# Autodesk Inventor assembly: gears
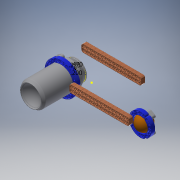
[picture p0: Inventor's stored thumbnail of the model, 180x180]
Saved by Autodesk Inventor 2019.3 (Build 233278000, 278)
## iProperties
Created: 2019-01-24
Part Number: gears
Document SubType Name: Assembly
Designer: Varga Daniel
Author: Varga Daniel
## Documents named in this file (9)
- C:\!_Dani\!_cloud\OneDrive\!_munka\Revolution\RevvyDemoKit\Structural parts\Part_test_Assembly.iam
- C:\!_Dani\!_cloud\OneDrive\!_munka\Revolution\RevvyDemoKit\Structural parts\Beams\Straight Beams\S2+x2\S16x2.iam
- C:\!_Dani\!_cloud\OneDrive\!_munka\Revolution\RevvyDemoKit\Structural parts\Beams\Straight Beams\S2+x2.iam
- C:\!_Dani\!_cloud\OneDrive\!_munka\Revolution\RevvyDemoKit\Structural parts\Beams\Curved beams\CB4H.ipt
- C:\!_Dani\!_cloud\OneDrive\!_munka\Revolution\RevvyDemoKit\Structural parts\Beams\Curved beams\CB6H.ipt
- C:\!_Dani\!_cloud\OneDrive\!_munka\Revolution\RevvyDemoKit\Structural parts\Beams\Curved beams\cocacola can.ipt
- C:\!_Dani\!_cloud\OneDrive\!_munka\Revolution\RevvyDemoKit\Structural parts\Beams\Straight Beams\S2+x1\S2x1.iam
- C:\!_Dani\!_cloud\OneDrive\!_munka\Revolution\RevvyDemoKit\Structural parts\Beams\Straight Beams\S2+x1.iam
- C:\!_Dani\!_cloud\OneDrive\!_munka\Revolution\RevvyDemoKit\Structural parts\Beams\Curved beams\Table tennis ball.ipt
## Components (14 placed, 6 different names)
1. S16x2:1 [sub-assembly] — Mate:1, Mate:2, Mate:3, Mate:4, Mate:14, Mate:15, Mate:16, Mate:17, Mate:25, Mate:26
2. S16x2:2 [sub-assembly]
3. CB4H:1 — Mate:14, Mate:15, Mate:19, Mate:26, Tangent:1
4. CB6H:1 — Mate:1, Mate:2, Mate:6, Mate:12, Mate:13
5. cocacola can:1 — Mate:5, Flush:1, Mate:6, Mate:11
6. CB6H:2 — Mate:3, Mate:4, Mate:5, Flush:1, Mate:9, Mate:10
7. S2x1:1 [sub-assembly] — Mate:7, Mate:8, Mate:9, Mate:10
8. S2x1:2 [sub-assembly] — Mate:12, Mate:13, Tangent:2
9. S2x1:3 [sub-assembly] — Mate:22, Mate:23, Mate:24
10. CB6H:3 — Mate:7, Mate:8, Mate:11, Tangent:2
11. Table tennis ball:1 — Mate:18, Mate:19, Mate:20, Mate:21
12. CB4H:2 — Mate:16, Mate:17, Mate:18, Mate:21, Flush:2, Mate:22, Mate:23, Mate:25
13. CB4H:3 — Mate:20, Flush:2, Mate:24, Mate:27, Mate:28
14. S2x1:4 [sub-assembly] — Mate:27, Mate:28, Tangent:1
## Relationships (32: Mate 28, Flush 2, Tangent 2)
- Mate:1: S16x2:1 ↔ CB6H:1
- Mate:2: S16x2:1 ↔ CB6H:1
- Mate:3: S16x2:1 ↔ CB6H:2
- Mate:4: S16x2:1 ↔ CB6H:2
- Mate:5: cocacola can:1 ↔ CB6H:2
- Flush:1 (-30 mm): cocacola can:1 ↔ CB6H:2
- Mate:6: CB6H:1 ↔ cocacola can:1
- Mate:7: S2x1:1 ↔ CB6H:3
- Mate:8: S2x1:1 ↔ CB6H:3
- Mate:9: CB6H:2 ↔ S2x1:1
- Mate:10: CB6H:2 ↔ S2x1:1
- Mate:11: cocacola can:1 ↔ CB6H:3
- Mate:12: CB6H:1 ↔ S2x1:2
- Mate:13: CB6H:1 ↔ S2x1:2
- Mate:14: S16x2:1 ↔ CB4H:1
- Mate:15: S16x2:1 ↔ CB4H:1
- Mate:16: S16x2:1 ↔ CB4H:2
- Mate:17: S16x2:1 ↔ CB4H:2
- Mate:18: Table tennis ball:1 ↔ CB4H:2
- Mate:19: CB4H:1 ↔ Table tennis ball:1
- Mate:20: Table tennis ball:1 ↔ CB4H:3
- Mate:21: Table tennis ball:1 ↔ CB4H:2
- Flush:2: CB4H:2 ↔ CB4H:3
- Mate:22: S2x1:3 ↔ CB4H:2
- Mate:23: S2x1:3 ↔ CB4H:2
- Mate:24: S2x1:3 ↔ CB4H:3
- Mate:25: S16x2:1 ↔ CB4H:2
- Mate:26: S16x2:1 ↔ CB4H:1
- Mate:27: CB4H:3 ↔ S2x1:4
- Mate:28: CB4H:3 ↔ S2x1:4
- Tangent:1: CB4H:1 ↔ S2x1:4
- Tangent:2: S2x1:2 ↔ CB6H:3
